# Autodesk Inventor assembly: cellSTORM_v5
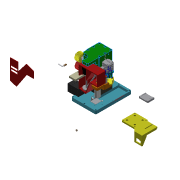
[picture p0: Inventor's stored thumbnail of the model, 180x180]
Saved by Autodesk Inventor 2022 (Build 260153000, 153)
## iProperties
Created: 2020-04-25
Part Number: cellSTORM_v5
Document SubType Name: Assembly
Designer: diederichbenedict
Author: diederichbenedict
## Documents named in this file (20)
- C:\Users\Muriel\Documents\GitHub\cellstorm\INVENTOR\cellSTORM_v6.iam
- C:\Users\Muriel\Documents\GitHub\cellstorm\INVENTOR\00_XY_stage-CHUO_SEIKI_LD-647-R1.iam
- C:\Users\Muriel\Documents\GitHub\cellstorm\INVENTOR\cellSTORM_laserbeam.ipt
- C:\Users\Muriel\Documents\GitHub\cellstorm\INVENTOR\00_Ballmagnets_5mm.ipt
- C:\Users\Muriel\Documents\GitHub\cellstorm\INVENTOR\00_Huawei_P20.ipt
- C:\Users\Muriel\Documents\GitHub\cellstorm\INVENTOR\cellSTORM_Base_v0_R1.ipt
- C:\Users\Muriel\Documents\GitHub\cellstorm\INVENTOR\00_KES400.iam
- C:\Users\Muriel\Documents\GitHub\cellstorm\INVENTOR\cellSTORM_v5_laserstage.ipt
- C:\Users\Muriel\Documents\GitHub\cellstorm\INVENTOR\cellSTORM_v5_cellphonestage.ipt
- C:\Users\Muriel\Documents\GitHub\cellstorm\INVENTOR\cellSTORM_v5_microsocpe.iam
- C:\Users\Muriel\Documents\GitHub\cellstorm\INVENTOR\cellSTORM_v5_microscope_cover.ipt
- C:\Users\Muriel\Documents\GitHub\cellstorm\INVENTOR\00_chip_01_old.ipt
- C:\Users\Muriel\Documents\GitHub\cellstorm\INVENTOR\cellSTORM_v5_chiptray_old_0.ipt
- C:\Users\Muriel\Documents\GitHub\cellstorm\INVENTOR\00_Laser_532nm_200mw.ipt
- C:\Users\Muriel\Documents\GitHub\cellstorm\INVENTOR\00_LN680-Step.ipt
- C:\Users\Muriel\Documents\GitHub\cellstorm\INVENTOR\cellSTORM_v5_motorblock.ipt
- C:\Users\Muriel\Documents\GitHub\cellstorm\INVENTOR\Assembly_Nema_Motor_attachement_for_XYstage.iam
- C:\Users\Muriel\Documents\GitHub\cellstorm\INVENTOR\00_Arduino_CNC_Assembly.iam
- C:\Users\Muriel\Documents\GitHub\cellstorm\INVENTOR\00_LASER_640nm.ipt
- C:\Users\diederichbenedict\Dropbox\cellSTORM\cellSTORM_v6.iam
## Components (22 placed, 18 different names)
1. 00_XY_stage-CHUO_SEIKI_LD-647-R1:1 [sub-assembly] — Insert:1, Angle:1, Insert:6, Angle:5
2. cellSTORM_laserbeam:1 — Passend:25
3. 00_Ballmagnets_5mm:1
4. 00_Ballmagnets_5mm:2
5. 00_Ballmagnets_5mm:3
6. cellSTORM_Base_v0_R1:1 — Insert:1, Angle:1, Winkel:7, Passend:27
7. 00_XY_stage-CHUO_SEIKI_LD-647-R1:2 [sub-assembly] — Insert:6, Angle:5, Flush:12, Flush:13, Insert:17, Mate:26
8. cellSTORM_v5_cellphonestage:1 — Flush:12, Flush:13, Flush:29, Fluchtend:33, Fluchtend:34, Fluchtend:35, Passend:29
9. cellSTORM_v5_microscope_cover:1
10. 00_Huawei_P20:1
11. 00_Laser_532nm_200mw:1 — Passend:25
12. 00_LN680-Step:1
13. cellSTORM_v5_motorblock:1 — Flush:29
14. Assembly_Nema_Motor_attachement_for_XYstage:1 [sub-assembly] — Insert:17
15. Assembly_Nema_Motor_attachement_for_XYstage:2 [sub-assembly] — Mate:26
16. 00_Arduino_CNC_Assembly:1 [sub-assembly] — Fluchtend:33, Fluchtend:34, Fluchtend:35
17. cellSTORM_v5_laserstage:1
18. 00_LASER_640nm:1 — Passend:28, Winkel:8
19. cellSTORM_v5_chiptray_old_0:1
20. 00_KES400:1 [sub-assembly] — Einfügen:18, Winkel:6, Passend:28
21. 00_chip_01_old:1 — Einfügen:18, Winkel:6, Winkel:7, Passend:27, Winkel:8
22. cellSTORM_v5_microsocpe:1 [sub-assembly] — Passend:29
## Relationships (20: Flush 6, Angle 5, Mate 5, Insert 4)
- Insert:1: 00_XY_stage-CHUO_SEIKI_LD-647-R1:1 ↔ cellSTORM_Base_v0_R1:1
- Angle:1 (90 deg): 00_XY_stage-CHUO_SEIKI_LD-647-R1:1 ↔ cellSTORM_Base_v0_R1:1
- Insert:6 (6 mm): 00_XY_stage-CHUO_SEIKI_LD-647-R1:1 ↔ 00_XY_stage-CHUO_SEIKI_LD-647-R1:2
- Angle:5 (180 deg): 00_XY_stage-CHUO_SEIKI_LD-647-R1:1 ↔ 00_XY_stage-CHUO_SEIKI_LD-647-R1:2
- Flush:12: 00_XY_stage-CHUO_SEIKI_LD-647-R1:2 ↔ cellSTORM_v5_cellphonestage:1
- Flush:13: 00_XY_stage-CHUO_SEIKI_LD-647-R1:2 ↔ cellSTORM_v5_cellphonestage:1
- Passend:25 [Mate]: cellSTORM_laserbeam:1 ↔ 00_Laser_532nm_200mw:1
- Flush:29: cellSTORM_v5_cellphonestage:1 ↔ cellSTORM_v5_motorblock:1
- Insert:17 (10 mm): 00_XY_stage-CHUO_SEIKI_LD-647-R1:2 ↔ Assembly_Nema_Motor_attachement_for_XYstage:1
- Mate:26 (5 mm): 00_XY_stage-CHUO_SEIKI_LD-647-R1:2 ↔ Assembly_Nema_Motor_attachement_for_XYstage:2
- Fluchtend:33 [Flush] (12 mm): cellSTORM_v5_cellphonestage:1 ↔ 00_Arduino_CNC_Assembly:1
- Fluchtend:34 [Flush] (-3 mm): cellSTORM_v5_cellphonestage:1 ↔ 00_Arduino_CNC_Assembly:1
- Fluchtend:35 [Flush] (5 mm): cellSTORM_v5_cellphonestage:1 ↔ 00_Arduino_CNC_Assembly:1
- Einfügen:18 [Insert] (1 mm): 00_KES400:1 ↔ 00_chip_01_old:1
- Winkel:6 [Angle] (0 deg): 00_KES400:1 ↔ 00_chip_01_old:1
- Winkel:7 [Angle] (0 deg): cellSTORM_Base_v0_R1:1 ↔ 00_chip_01_old:1
- Passend:27 [Mate] (13 mm): cellSTORM_Base_v0_R1:1 ↔ 00_chip_01_old:1
- Passend:28 [Mate]: 00_LASER_640nm:1 ↔ 00_KES400:1
- Winkel:8 [Angle] (0 deg): 00_LASER_640nm:1 ↔ 00_chip_01_old:1
- Passend:29 [Mate]: cellSTORM_v5_cellphonestage:1 ↔ cellSTORM_v5_microsocpe:1
